# Autodesk Inventor assembly: PataMesa
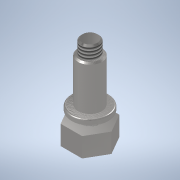
[picture p0: Inventor's stored thumbnail of the model, 180x180]
Saved by Autodesk Inventor 2020.3 (Build 243373010, 373A)
## iProperties
Created: 2020-11-11
Part Number: PataMesa
Document SubType Name: Assembly
Designer: codig
Author: codig
## Documents named in this file (4)
- C:\Users\codig\Documents\GrabCAD\EscritorioV4\PataMesa\PataMesa.iam
- C:\Users\codig\Documents\GrabCAD\EscritorioV4\PataMesa\Pieza1.ipt
- C:\Users\codig\Documents\GrabCAD\EscritorioV4\PataMesa\Pieza1.1.ipt
- C:\Users\codig\Documents\GrabCAD\EscritorioV4\PataMesa\Pieza2.ipt
## Components (3 placed, 3 different names)
1. Pieza1:1 — Rígido:1
2. Pieza1.1:1 — Rígido:1, Cilíndrica:1
3. Pieza2:1 — Cilíndrica:1
## Relationships (2: WeldJoint 1, CylindricalJoint 1)
- Rígido:1 [WeldJoint]: Pieza1:1 ↔ Pieza1.1:1
- Cilíndrica:1 [CylindricalJoint]: Pieza1.1:1 ↔ Pieza2:1
